# Autodesk Inventor assembly: 200-40-BOGIE-CONNECTOR-ASM-01
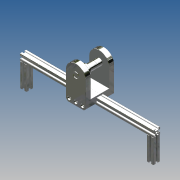
[picture p0: Inventor's stored thumbnail of the model, 180x180]
Saved by Autodesk Inventor 2018.2 (Build 222227000, 227)
## iProperties
Manager: feesmrt
Company: FRANC0R
Created: 2017-12-10
Part Number: 200-40-BOGIE-CONNECTOR-ASM-01
Material: Generisch
Document SubType Name: Assembly
Designer: feesmrt
Project: Rescue Robot
Cost Center: -
Description: Bogie Connector Assembly
Engineer: feesmrt
Authority: feesmrt
Stock Number: 200-40-BOGIE-CONNECTOR-ASM-01
Author: feesmrt
Title: Bogie Connector Assembly
Subject: Rescue Robot
Revision Number: 1
## Documents named in this file (6)
- D:\Programmierung\FRANC0R\CAD\02-Rocker-Bogie-Robot\200-ROCKER-BOGIE\200-40-BOGIE-CONNECTOR-ASM-01.iam
- D:\Programmierung\FRANC0R\CAD\02-Rocker-Bogie-Robot\900-COMPONENTS\900-50-PROFILES\90-50-PROFILES-20x20x400.ipt
- D:\Programmierung\FRANC0R\CAD\02-Rocker-Bogie-Robot\900-COMPONENTS\900-50-PROFILES\90-50-PROFILES-20x20x70.ipt
- D:\Programmierung\FRANC0R\CAD\02-Rocker-Bogie-Robot\200-ROCKER-BOGIE\200-40-BOGIE-CONNECTOR-05.ipt
- D:\Programmierung\FRANC0R\CAD\02-Rocker-Bogie-Robot\200-ROCKER-BOGIE\200-40-BOGIE-CONNECTOR-03.ipt
- D:\Programmierung\FRANC0R\CAD\02-Rocker-Bogie-Robot\200-ROCKER-BOGIE\200-40-BOGIE-CONNECTOR-04.ipt
## Components (8 placed, 5 different names)
1. 200-40-BOGIE-CONNECTOR-05:1 — Passend:6, Passend:7, Fluchtend:7, Passend:8, Passend:9, Passend:10
2. 200-40-BOGIE-CONNECTOR-03:2 — Passend:8, Passend:9, Passend:10, Passend:14, Passend:16, Passend:20
3. 200-40-BOGIE-CONNECTOR-03:1 — Passend:6, Passend:7, Fluchtend:7, Passend:17, Passend:18, Passend:19
4. 90-50-PROFILES-20x20x400:1 — Passend:4, Fluchtend:3, Fluchtend:4, Passend:5, Fluchtend:5, Fluchtend:6, Fluchtend:9, Passend:21, Passend:22
5. 90-50-PROFILES-20x20x70:1 — Passend:5, Fluchtend:5, Fluchtend:6
6. 90-50-PROFILES-20x20x70:2 — Passend:4, Fluchtend:3, Fluchtend:4
7. 200-40-BOGIE-CONNECTOR-04:1 — Passend:17, Passend:18, Passend:19, Passend:21
8. 200-40-BOGIE-CONNECTOR-04:2 — Passend:14, Passend:16, Passend:20, Passend:22
## Relationships (21: Mate 15, Flush 6)
- Passend:4 [Mate]: 90-50-PROFILES-20x20x400:1 ↔ 90-50-PROFILES-20x20x70:2
- Fluchtend:3 [Flush]: 90-50-PROFILES-20x20x400:1 ↔ 90-50-PROFILES-20x20x70:2
- Fluchtend:4 [Flush]: 90-50-PROFILES-20x20x400:1 ↔ 90-50-PROFILES-20x20x70:2
- Passend:5 [Mate]: 90-50-PROFILES-20x20x400:1 ↔ 90-50-PROFILES-20x20x70:1
- Fluchtend:5 [Flush]: 90-50-PROFILES-20x20x400:1 ↔ 90-50-PROFILES-20x20x70:1
- Fluchtend:6 [Flush]: 90-50-PROFILES-20x20x400:1 ↔ 90-50-PROFILES-20x20x70:1
- Passend:6 [Mate]: 200-40-BOGIE-CONNECTOR-05:1 ↔ 200-40-BOGIE-CONNECTOR-03:1
- Passend:7 [Mate]: 200-40-BOGIE-CONNECTOR-05:1 ↔ 200-40-BOGIE-CONNECTOR-03:1
- Fluchtend:7 [Flush]: 200-40-BOGIE-CONNECTOR-05:1 ↔ 200-40-BOGIE-CONNECTOR-03:1
- Passend:8 [Mate]: 200-40-BOGIE-CONNECTOR-05:1 ↔ 200-40-BOGIE-CONNECTOR-03:2
- Passend:9 [Mate]: 200-40-BOGIE-CONNECTOR-05:1 ↔ 200-40-BOGIE-CONNECTOR-03:2
- Passend:10 [Mate]: 200-40-BOGIE-CONNECTOR-05:1 ↔ 200-40-BOGIE-CONNECTOR-03:2
- Passend:14 [Mate]: 200-40-BOGIE-CONNECTOR-03:2 ↔ 200-40-BOGIE-CONNECTOR-04:2
- Passend:16 [Mate]: 200-40-BOGIE-CONNECTOR-03:2 ↔ 200-40-BOGIE-CONNECTOR-04:2
- Fluchtend:9 [Flush]: 90-50-PROFILES-20x20x400:1
- Passend:17 [Mate]: 200-40-BOGIE-CONNECTOR-03:1 ↔ 200-40-BOGIE-CONNECTOR-04:1
- Passend:18 [Mate]: 200-40-BOGIE-CONNECTOR-03:1 ↔ 200-40-BOGIE-CONNECTOR-04:1
- Passend:19 [Mate]: 200-40-BOGIE-CONNECTOR-03:1 ↔ 200-40-BOGIE-CONNECTOR-04:1
- Passend:20 [Mate]: 200-40-BOGIE-CONNECTOR-03:2 ↔ 200-40-BOGIE-CONNECTOR-04:2
- Passend:21 [Mate]: 90-50-PROFILES-20x20x400:1 ↔ 200-40-BOGIE-CONNECTOR-04:1
- Passend:22 [Mate]: 90-50-PROFILES-20x20x400:1 ↔ 200-40-BOGIE-CONNECTOR-04:2
